# Autodesk Inventor assembly: 3-2
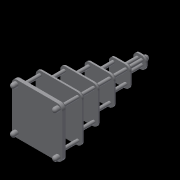
[picture p0: Inventor's stored thumbnail of the model, 180x180]
Saved by Autodesk Inventor 2017 (Build 210142000, 142)
## iProperties
Part Number: 3-2
Material: 一般
Document SubType Name: Assembly
Designer: r0909
Author: r0909
## Documents named in this file (9)
- C:\Users\r0909\Desktop\inventor\3-2.iam
- C:\Users\r0909\Desktop\inventor\2-5.ipt
- C:\Users\r0909\Desktop\inventor\2-6.ipt
- C:\Users\r0909\Desktop\inventor\2-7.ipt
- C:\Users\r0909\Desktop\inventor\3-1.2.ipt
- C:\Users\r0909\Desktop\inventor\3-1.3.ipt
- C:\Users\r0909\Desktop\inventor\3-1.4.ipt
- C:\Users\r0909\Desktop\inventor\3-1.5.ipt
- C:\Users\r0909\Desktop\inventor\3-1.6.ipt
## Components (31 placed, 8 different names)
1. 2-5:1 — 貼合:1, 貼合:2, 貼合:3, 貼合:4, 貼合:5, 貼合:6, 貼合:7, 貼合:8, 貼合:9, 貼合:10, 貼合:11, 貼合:12, 貼合:13, 貼合:14, 貼合:15, 貼合:16
2. 2-6:1 — 貼合:9, 貼合:10
3. 2-7:1 — 貼合:64, 貼合:65
4. 3-1.2:1 — 貼合:17, 貼合:18, 貼合:19, 貼合:20, 貼合:21, 貼合:22, 貼合:23, 貼合:24, 貼合:25, 貼合:26, 貼合:27
5. 3-1.3:1 — 貼合:28, 貼合:29, 貼合:30, 貼合:31, 貼合:32, 貼合:33, 貼合:34, 貼合:35, 貼合:36, 貼合:37, 貼合:38
6. 3-1.4:1 — 貼合:39, 貼合:40, 貼合:41, 貼合:42, 貼合:43, 貼合:44, 貼合:45, 貼合:46, 貼合:47, 貼合:48, 貼合:49
7. 3-1.5:1 — 貼合:50, 貼合:51, 貼合:52, 貼合:53, 貼合:54, 貼合:55, 貼合:56, 貼合:57, 貼合:58, 貼合:59, 貼合:60
8. 3-1.6:1 — 貼合:61, 貼合:62, 貼合:63, 貼合:64, 貼合:65
9. 2-7:2 — 貼合:2, 貼合:7
10. 2-7:3 — 貼合:1, 貼合:5
11. 2-7:4 — 貼合:3, 貼合:8
12. 2-7:5 — 貼合:4, 貼合:6
13. 2-6:2 — 貼合:13, 貼合:16, 貼合:17
14. 2-6:3 — 貼合:12, 貼合:15
15. 2-6:4 — 貼合:11, 貼合:14, 貼合:18, 貼合:19
16. 2-6:5 — 貼合:20, 貼合:24
17. 2-6:6 — 貼合:21, 貼合:25
18. 2-6:7 — 貼合:22, 貼合:26, 貼合:29, 貼合:30
19. 2-6:8 — 貼合:23, 貼合:27, 貼合:28
20. 2-6:9 — 貼合:32, 貼合:37, 貼合:39, 貼合:41
21. 2-6:10 — 貼合:33, 貼合:38
22. 2-6:11 — 貼合:34, 貼合:36, 貼合:40
23. 2-6:12 — 貼合:31, 貼合:35
24. 2-6:13 — 貼合:45, 貼合:47, 貼合:50
25. 2-6:14 — 貼合:43, 貼合:46
26. 2-6:15 — 貼合:44, 貼合:49
27. 2-6:16 — 貼合:42, 貼合:48, 貼合:51, 貼合:52
28. 2-6:17 — 貼合:53, 貼合:58, 貼合:61
29. 2-6:18 — 貼合:54, 貼合:57
30. 2-6:19 — 貼合:55, 貼合:59
31. 2-6:20 — 貼合:56, 貼合:60, 貼合:62, 貼合:63
## Relationships (65: Mate 65)
- 貼合:1 [Mate]: 2-5:1 ↔ 2-7:3
- 貼合:2 [Mate]: 2-5:1 ↔ 2-7:2
- 貼合:3 [Mate]: 2-5:1 ↔ 2-7:4
- 貼合:4 [Mate]: 2-5:1 ↔ 2-7:5
- 貼合:5 [Mate]: 2-5:1 ↔ 2-7:3
- 貼合:6 [Mate]: 2-5:1 ↔ 2-7:5
- 貼合:7 [Mate]: 2-5:1 ↔ 2-7:2
- 貼合:8 [Mate]: 2-5:1 ↔ 2-7:4
- 貼合:9 [Mate]: 2-5:1 ↔ 2-6:1
- 貼合:10 [Mate]: 2-5:1 ↔ 2-6:1
- 貼合:11 [Mate]: 2-5:1 ↔ 2-6:4
- 貼合:12 [Mate]: 2-5:1 ↔ 2-6:3
- 貼合:13 [Mate]: 2-5:1 ↔ 2-6:2
- 貼合:14 [Mate]: 2-5:1 ↔ 2-6:4
- 貼合:15 [Mate]: 2-5:1 ↔ 2-6:3
- 貼合:16 [Mate]: 2-5:1 ↔ 2-6:2
- 貼合:17 [Mate]: 3-1.2:1 ↔ 2-6:2
- 貼合:18 [Mate]: 3-1.2:1 ↔ 2-6:4
- 貼合:19 [Mate]: 3-1.2:1 ↔ 2-6:4
- 貼合:20 [Mate]: 3-1.2:1 ↔ 2-6:5
- 貼合:21 [Mate]: 3-1.2:1 ↔ 2-6:6
- 貼合:22 [Mate]: 3-1.2:1 ↔ 2-6:7
- 貼合:23 [Mate]: 3-1.2:1 ↔ 2-6:8
- 貼合:24 [Mate]: 3-1.2:1 ↔ 2-6:5
- 貼合:25 [Mate]: 3-1.2:1 ↔ 2-6:6
- 貼合:26 [Mate]: 3-1.2:1 ↔ 2-6:7
- 貼合:27 [Mate]: 3-1.2:1 ↔ 2-6:8
- 貼合:28 [Mate]: 3-1.3:1 ↔ 2-6:8
- 貼合:29 [Mate]: 3-1.3:1 ↔ 2-6:7
- 貼合:30 [Mate]: 3-1.3:1 ↔ 2-6:7
- 貼合:31 [Mate]: 3-1.3:1 ↔ 2-6:12
- 貼合:32 [Mate]: 3-1.3:1 ↔ 2-6:9
- 貼合:33 [Mate]: 3-1.3:1 ↔ 2-6:10
- 貼合:34 [Mate]: 3-1.3:1 ↔ 2-6:11
- 貼合:35 [Mate]: 3-1.3:1 ↔ 2-6:12
- 貼合:36 [Mate]: 3-1.3:1 ↔ 2-6:11
- 貼合:37 [Mate]: 3-1.3:1 ↔ 2-6:9
- 貼合:38 [Mate]: 3-1.3:1 ↔ 2-6:10
- 貼合:39 [Mate]: 3-1.4:1 ↔ 2-6:9
- 貼合:40 [Mate]: 3-1.4:1 ↔ 2-6:11
- 貼合:41 [Mate]: 3-1.4:1 ↔ 2-6:9
- 貼合:42 [Mate]: 3-1.4:1 ↔ 2-6:16
- 貼合:43 [Mate]: 3-1.4:1 ↔ 2-6:14
- 貼合:44 [Mate]: 3-1.4:1 ↔ 2-6:15
- 貼合:45 [Mate]: 3-1.4:1 ↔ 2-6:13
- 貼合:46 [Mate]: 3-1.4:1 ↔ 2-6:14
- 貼合:47 [Mate]: 3-1.4:1 ↔ 2-6:13
- 貼合:48 [Mate]: 3-1.4:1 ↔ 2-6:16
- 貼合:49 [Mate]: 3-1.4:1 ↔ 2-6:15
- 貼合:50 [Mate]: 3-1.5:1 ↔ 2-6:13
- 貼合:51 [Mate]: 3-1.5:1 ↔ 2-6:16
- 貼合:52 [Mate]: 3-1.5:1 ↔ 2-6:16
- 貼合:53 [Mate]: 3-1.5:1 ↔ 2-6:17
- 貼合:54 [Mate]: 3-1.5:1 ↔ 2-6:18
- 貼合:55 [Mate]: 3-1.5:1 ↔ 2-6:19
- 貼合:56 [Mate]: 3-1.5:1 ↔ 2-6:20
- 貼合:57 [Mate]: 3-1.5:1 ↔ 2-6:18
- 貼合:58 [Mate]: 3-1.5:1 ↔ 2-6:17
- 貼合:59 [Mate]: 3-1.5:1 ↔ 2-6:19
- 貼合:60 [Mate]: 3-1.5:1 ↔ 2-6:20
- 貼合:61 [Mate]: 3-1.6:1 ↔ 2-6:17
- 貼合:62 [Mate]: 3-1.6:1 ↔ 2-6:20
- 貼合:63 [Mate]: 3-1.6:1 ↔ 2-6:20
- 貼合:64 [Mate]: 2-7:1 ↔ 3-1.6:1
- 貼合:65 [Mate]: 2-7:1 ↔ 3-1.6:1
